# Autodesk Inventor assembly: Birdhouse Assembly 1
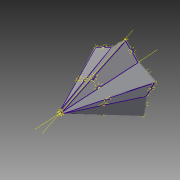
[picture p0: Inventor's stored thumbnail of the model, 180x180]
Saved by Autodesk Inventor 2015 (Build 190159000, 159)
## iProperties
Created: 2018-03-08
Part Number: Birdhouse Assembly 1
Document SubType Name: Assembly
Designer: Administrator
Author: Administrator
## Documents named in this file (4)
- L:\IED 9th\Birdhouse Assembly 1.iam
- L:\IED 9th\Star Base.ipt
- L:\IED 9th\Star Side Out.ipt
- L:\IED 9th\Star Side.ipt
## Components (11 placed, 3 different names)
1. Star Base:1 — Mate:2, Mate:3, Mate:7, Mate:8, Mate:12, Mate:13, Mate:16, Mate:17, Mate:21, Mate:24, Mate:25, Mate:26, Mate:27, Mate:28, Mate:30, Mate:31, Mate:32, Mate:33, Mate:34, Mate:35
2. Star Side Out:1 — Mate:2, Mate:3
3. Star Side Out:2 — Mate:7, Mate:8
4. Star Side Out:3 — Mate:12, Mate:13
5. Star Side Out:4 — Mate:16, Mate:17
6. Star Side Out:5 — Mate:21, Mate:24
7. Star Side:1 — Mate:27, Mate:28
8. Star Side:2 — Mate:25, Mate:26
9. Star Side:3 — Mate:32, Mate:33
10. Star Side:4 — Mate:34, Mate:35
11. Star Side:5 — Mate:30, Mate:31
## Relationships (20: Mate 20)
- Mate:2: Star Base:1 ↔ Star Side Out:1
- Mate:3: Star Base:1 ↔ Star Side Out:1
- Mate:7: Star Base:1 ↔ Star Side Out:2
- Mate:8: Star Base:1 ↔ Star Side Out:2
- Mate:12: Star Base:1 ↔ Star Side Out:3
- Mate:13: Star Base:1 ↔ Star Side Out:3
- Mate:16: Star Base:1 ↔ Star Side Out:4
- Mate:17: Star Base:1 ↔ Star Side Out:4
- Mate:21: Star Base:1 ↔ Star Side Out:5
- Mate:24: Star Base:1 ↔ Star Side Out:5
- Mate:25: Star Base:1 ↔ Star Side:2
- Mate:26: Star Base:1 ↔ Star Side:2
- Mate:27: Star Base:1 ↔ Star Side:1
- Mate:28: Star Base:1 ↔ Star Side:1
- Mate:30: Star Base:1 ↔ Star Side:5
- Mate:31: Star Base:1 ↔ Star Side:5
- Mate:32: Star Base:1 ↔ Star Side:3
- Mate:33: Star Base:1 ↔ Star Side:3
- Mate:34: Star Base:1 ↔ Star Side:4
- Mate:35: Star Base:1 ↔ Star Side:4
